# Autodesk Inventor assembly: ASY PNS 1662 FDS way 2
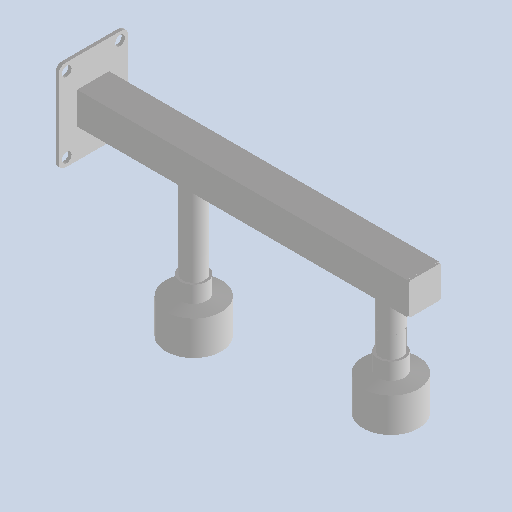
[picture p0: Inventor's stored thumbnail of the model, 512x512]
Saved by Autodesk Inventor 2025 (Build 290162010, 162A)
## iProperties
Created: 2025-07-02
Part Number: ASY PNS 1662 FDS way 2
Document SubType Name: Assembly
Designer: admin
Author: user
## Documents named in this file (8)
- C:\Users\pokla\Documents\Inventor\PNS2-Panaevsk\Filter D1000\filter-distribution-system 1000\ASY PNS 1662 FDS way 2.iam
- C:\Users\pokla\Documents\Inventor\PNS2-Panaevsk\Filter D1000\filter-distribution-system 1000\PNS 1662 FDS 1000 way tube 2.ipt
- C:\Users\pokla\Documents\Inventor\PNS2-Panaevsk\Filter D1000\filter-distribution-system 1000\PNS dummy filter element_1600.ipt
- C:\Users\pokla\Documents\Inventor\PNS2-Panaevsk\Filter D1000\filter-distribution-system 1000\PNS dummy pipe nippel_1600.ipt
- C:\Users\pokla\Documents\Inventor\PNS2-Panaevsk\Filter D1000\filter-distribution-system 1000\PNS 1686 FDS 1000 way tube 6.ipt
- C:\Users\pokla\Documents\Inventor\PNS2-Panaevsk\Filter D1000\filter-distribution-system 1000\PNS 1687 FDS 1000 way tube 7.ipt
- C:\Users\pokla\Documents\Inventor\PNS2-Panaevsk\Filter D1000\filter-distribution-system 1000\PNS 1669 FDS 1000 FLANGE 3.ipt
- C:\Users\pokla\Documents\Inventor\PNS2-Panaevsk\Filter D1000\filter-distribution-system 1000\PNS 1666 FDS 1000 CUP 1.ipt
## Components (9 placed, 7 different names)
1. PNS 1662 FDS 1000 way tube 2.ipt:1 — Rigid:5, Rigid:8, Rigid:9, Rigid:10
2. PNS 1686 FDS 1000 way tube 6.ipt:1 — Rigid:5, Rigid:4
3. PNS dummy filter element_1600.ipt:2 — Rigid:3
4. PNS dummy pipe nippel_1600.ipt:2 — Rigid:4, Rigid:3
5. PNS 1687 FDS 1000 way tube 7.ipt:1 — Rigid:8, Rigid:7
6. PNS dummy filter element_1600.ipt:3 — Rigid:6
7. PNS dummy pipe nippel_1600.ipt:3 — Rigid:7, Rigid:6
8. PNS 1669 FDS 1000 FLANGE 3.ipt:1 — Rigid:9
9. PNS 1666 FDS 1000 CUP 1.ipt:1 — Rigid:10
## Relationships (8: WeldJoint 8)
- Rigid:5 [WeldJoint]: PNS 1662 FDS 1000 way tube 2.ipt:1 ↔ PNS 1686 FDS 1000 way tube 6.ipt:1
- Rigid:4 [WeldJoint]: PNS 1686 FDS 1000 way tube 6.ipt:1 ↔ PNS dummy pipe nippel_1600.ipt:2
- Rigid:3 [WeldJoint]: PNS dummy filter element_1600.ipt:2 ↔ PNS dummy pipe nippel_1600.ipt:2
- Rigid:8 [WeldJoint]: PNS 1662 FDS 1000 way tube 2.ipt:1 ↔ PNS 1687 FDS 1000 way tube 7.ipt:1
- Rigid:7 [WeldJoint]: PNS 1687 FDS 1000 way tube 7.ipt:1 ↔ PNS dummy pipe nippel_1600.ipt:3
- Rigid:6 [WeldJoint]: PNS dummy filter element_1600.ipt:3 ↔ PNS dummy pipe nippel_1600.ipt:3
- Rigid:9 [WeldJoint] (-3 mm): PNS 1662 FDS 1000 way tube 2.ipt:1 ↔ PNS 1669 FDS 1000 FLANGE 3.ipt:1
- Rigid:10 [WeldJoint]: PNS 1662 FDS 1000 way tube 2.ipt:1 ↔ PNS 1666 FDS 1000 CUP 1.ipt:1
